# Autodesk Inventor assembly: robot4
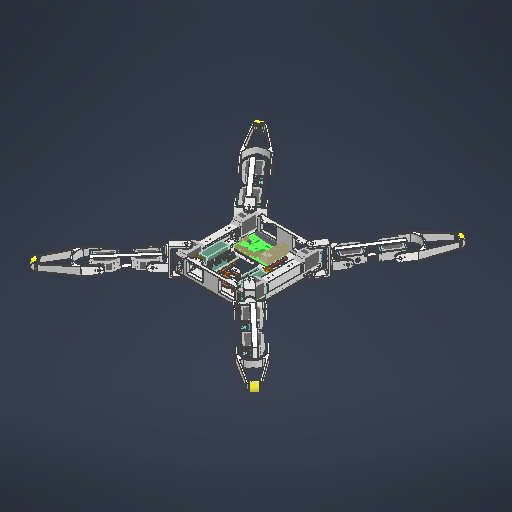
[picture p0: Inventor's stored thumbnail of the model, 512x512]
Saved by Autodesk Inventor 2026.1 (Build 301233000, 233)
## iProperties
Created: 2025-11-03
Part Number: robot4
Document SubType Name: Assembly
Designer: emanuel
Author: emanuel
## Documents named in this file (22)
- C:\Users\emanuel\UnFolder\SpiderRobo\3dmodel\robot6.iam
- C:\Users\emanuel\UnFolder\SpiderRobo\3dmodel\rigid_support1.ipt
- C:\Users\emanuel\UnFolder\SpiderRobo\3dmodel\mg996r.ipt
- C:\Users\emanuel\UnFolder\SpiderRobo\3dmodel\servo_support_4.ipt
- C:\Users\emanuel\UnFolder\SpiderRobo\3dmodel\servo_disc.ipt
- C:\Users\emanuel\UnFolder\SpiderRobo\3dmodel\C1.ipt
- C:\Users\emanuel\UnFolder\SpiderRobo\3dmodel\back_plate.ipt
- C:\Users\emanuel\UnFolder\SpiderRobo\3dmodel\smart_calf.ipt
- C:\Users\emanuel\UnFolder\SpiderRobo\3dmodel\back_servo_support.ipt
- C:\Users\emanuel\UnFolder\SpiderRobo\3dmodel\C2.ipt
- C:\Users\emanuel\UnFolder\SpiderRobo\3dmodel\femur.ipt
- C:\Users\emanuel\UnFolder\SpiderRobo\3dmodel\shoe.ipt
- C:\Users\emanuel\UnFolder\SpiderRobo\3dmodel\shoe_lace.ipt
- C:\Users\emanuel\UnFolder\SpiderRobo\3dmodel\support_2_servo_wide.ipt
- C:\Users\emanuel\UnFolder\SpiderRobo\3dmodel\middle_base.ipt
- C:\Users\emanuel\UnFolder\SpiderRobo\3dmodel\servo_support_4_interior.ipt
- C:\Users\emanuel\UnFolder\SpiderRobo\3dmodel\side_wall1.ipt
- C:\Users\emanuel\UnFolder\SpiderRobo\3dmodel\side_wall2.ipt
- C:\Users\emanuel\UnFolder\SpiderRobo\3dmodel\servo_driver.ipt
- C:\Users\emanuel\UnFolder\SpiderRobo\3dmodel\electronics_holder3.ipt
- C:\Users\emanuel\UnFolder\SpiderRobo\3dmodel\electronics_holder.ipt
- C:\Users\emanuel\UnFolder\SpiderRobo\3dmodel\RaspberryPi5.ipt
## Components (92 placed, 21 different names)
1. rigid_support1:1 — Flush:7, Flush:18, Mate:299, Flush:28, Flush:42, Flush:43, Mate:352, Mate:357
2. rigid_support1:2 — Flush:7, Flush:19, Mate:303, Flush:29, Flush:38, Flush:39, Mate:353
3. mg996r:1 — Mate:7, Mate:8, Mate:20, Mate:21, Mate:251, Mate:301
4. servo_support_4:3 — Flush:1, Flush:3, Flush:24, Flush:25, Mate:301, Mate:342
5. servo_support_4:4 — Flush:1, Mate:7, Mate:8, Flush:26, Flush:27
6. mg996r:2 — Mate:22, Mate:23, Mate:257, Mate:302, Mate:343
7. servo_support_4:5 — Flush:22, Flush:23, Mate:302, Mate:344
8. servo_support_4:6 — Flush:3, Mate:300, Flush:20, Flush:21
9. servo_disc:1 — Mate:20, Mate:21, Mate:250
10. servo_disc:2 — Mate:22, Mate:23, Mate:256
11. mg996r:3 — Mate:247, Mate:298
12. servo_support_4:7 — Mate:298, Flush:32, Flush:36, Mate:339, Flush:47
13. servo_support_4:8 — Mate:304, Flush:30, Flush:31, Mate:321, Flush:44, Flush:45
14. mg996r:4 — Mate:249, Mate:297
15. servo_support_4:10 — Mate:297, Flush:35, Flush:37, Mate:322, Flush:46, Mate:323
16. servo_disc:3 — Mate:246
17. servo_disc:4 — Mate:248
18. back_plate:1
19. smart_calf:1 — Mate:128, Mate:129, Mate:273, Mate:274, Mate:275
20. servo_disc:7 — Mate:128
21. back_servo_support:3
22. C2:2 — Mate:130, Mate:131, Mate:132, Mate:133, Mate:134
23. femur:2
24. mg996r:7 — Mate:129
25. servo_disc:8
26. mg996r:8
27. back_servo_support:4
28. servo_support_4:16
29. servo_support_4:17
30. servo_support_4:18
31. servo_support_4:19
32. C1:1 — Mate:130, Mate:131, Mate:132, Mate:133, Mate:134, Mate:248, Mate:249
33. smart_calf:2 — Mate:289, Mate:290, Mate:291
34. servo_disc:9
35. back_servo_support:5
36. C2:3
37. femur:3
38. mg996r:9
39. servo_disc:10
40. mg996r:10
41. back_servo_support:6
42. servo_support_4:20
43. servo_support_4:21
44. servo_support_4:22
45. servo_support_4:23
46. C1:2 — Mate:256, Mate:257
47. smart_calf:3 — Mate:288, Mate:292, Mate:293
48. servo_disc:11
49. back_servo_support:7
50. C2:4
51. femur:4
52. mg996r:11
53. servo_disc:12
54. mg996r:12
55. back_servo_support:8
56. servo_support_4:24
57. servo_support_4:25
58. servo_support_4:26
59. servo_support_4:27
60. C1:3 — Mate:250, Mate:251
61. smart_calf:4 — Mate:285, Mate:286, Mate:287
62. servo_disc:13
63. back_servo_support:9
64. C2:5
65. femur:5
66. mg996r:13
67. servo_disc:14
68. mg996r:14
69. back_servo_support:10
70. servo_support_4:28
71. servo_support_4:29
72. servo_support_4:30
73. servo_support_4:31
74. C1:4 — Mate:246, Mate:247
75. shoe:1 — Mate:273, Mate:274, Mate:275, Mate:276, Mate:277, Mate:278
76. shoe_lace:1 — Mate:276, Mate:277, Mate:278
77. shoe:2 — Mate:285, Mate:286, Mate:287
78. shoe:3 — Mate:289, Mate:290, Mate:291
79. shoe:4 — Mate:288, Mate:292, Mate:293
80. support_2_servo_wide:2 — Flush:18, Flush:19, Mate:299, Mate:300, Flush:20, Flush:21, Flush:22, Flush:23, Flush:24, Flush:25, Flush:26, Flush:27
81. support_2_servo_wide:3 — Mate:303, Flush:28, Flush:29, Mate:304, Flush:30, Flush:31, Flush:32, Flush:35, Flush:36, Flush:37, Mate:305, Mate:306, Mate:307, Flush:38, Flush:39, Mate:314, Flush:40, Flush:41, Flush:42, Flush:43
82. middle_base:1 — Mate:305, Mate:306, Mate:307, Mate:354, Mate:355, Mate:356
83. servo_support_4_interior:1 — Mate:314, Flush:40, Flush:41, Mate:340, Mate:341
84. side_wall2:1 — Mate:321, Flush:44, Flush:45
85. side_wall2:2 — Mate:322, Flush:46, Mate:323
86. servo_driver:2 — Mate:349, Mate:350, Mate:351
87. servo_driver:3 — Mate:345, Mate:346, Mate:347, Mate:348
88. side_wall1:1 — Mate:339, Flush:47, Mate:340, Mate:341
89. side_wall1:2 — Mate:342, Mate:343, Mate:344
90. electronics_holder:1 — Mate:345, Mate:346, Mate:347, Mate:348, Mate:349, Mate:350, Mate:351, Mate:352, Mate:353, Mate:354
91. RaspberryPi5:1 — Mate:358, Mate:359, Mate:360
92. electronics_holder3:1 — Mate:355, Mate:356, Mate:357, Mate:358, Mate:359, Mate:360
## Relationships (258: Mate 224, Flush 34)
- Flush:1: servo_support_4:3 ↔ servo_support_4:4
- Mate:7: mg996r:1 ↔ servo_support_4:4
- Mate:8: mg996r:1 ↔ servo_support_4:4
- [Flush]: servo_support_4:5 ↔ servo_support_4:6
- [Mate]: mg996r:2 ↔ servo_support_4:6
- [Mate]: mg996r:2 ↔ servo_support_4:6
- Flush:3: servo_support_4:3 ↔ servo_support_4:6
- Mate:20: mg996r:1 ↔ servo_disc:1
- Mate:21: mg996r:1 ↔ servo_disc:1
- Mate:22: mg996r:2 ↔ servo_disc:2
- Mate:23: mg996r:2 ↔ servo_disc:2
- [Flush]: servo_support_4:7 ↔ servo_support_4:8
- [Mate]: mg996r:3 ↔ servo_support_4:8
- [Mate]: mg996r:3 ↔ servo_support_4:8
- [Mate]: mg996r:4 ↔ servo_support_4:10
- [Mate]: mg996r:4 ↔ servo_support_4:10
- [Flush]: servo_support_4:7 ↔ servo_support_4:10
- [Mate]: mg996r:3 ↔ servo_disc:3
- [Mate]: mg996r:3 ↔ servo_disc:3
- [Mate]: mg996r:4 ↔ servo_disc:4
- [Mate]: mg996r:4 ↔ servo_disc:4
- Flush:7: rigid_support1:1 ↔ rigid_support1:2
- [Mate]: servo_disc:7 ↔ mg996r:7
- [Mate]: servo_disc:7 ↔ mg996r:7
- [Mate]: servo_disc:8 ↔ mg996r:8
- [Mate]: servo_disc:8 ↔ mg996r:8
- [Mate]: femur:2 ↔ mg996r:8
- [Mate]: femur:2 ↔ mg996r:8
- [Mate]: femur:2 ↔ mg996r:8
- [Mate]: femur:2 ↔ mg996r:7
- [Mate]: femur:2 ↔ mg996r:7
- [Mate]: femur:2 ↔ mg996r:7
- [Mate]: C2:2 ↔ servo_disc:8
- [Mate]: C2:2 ↔ mg996r:8
- [Mate]: femur:2 ↔ servo_support_4:16
- [Mate]: femur:2 ↔ servo_support_4:19
- [Mate]: femur:2 ↔ servo_support_4:17
- [Mate]: femur:2 ↔ servo_support_4:18
- [Mate]: femur:2 ↔ servo_support_4:16
- [Mate]: mg996r:7 ↔ servo_support_4:19
- [Mate]: back_servo_support:4 ↔ servo_support_4:16
- [Mate]: back_servo_support:4 ↔ servo_support_4:16
- [Mate]: back_servo_support:4 ↔ servo_support_4:16
- [Mate]: back_servo_support:4 ↔ servo_support_4:19
- [Mate]: femur:2 ↔ servo_support_4:16
- [Mate]: femur:2 ↔ servo_support_4:18
- [Mate]: femur:2 ↔ servo_support_4:18
- [Mate]: mg996r:8 ↔ servo_support_4:17
- [Mate]: back_servo_support:3 ↔ servo_support_4:18
- [Mate]: back_servo_support:3 ↔ servo_support_4:18
- [Mate]: back_servo_support:3 ↔ servo_support_4:18
- [Mate]: back_servo_support:3 ↔ servo_support_4:17
- Mate:128: smart_calf:1 ↔ servo_disc:7
- Mate:129: smart_calf:1 ↔ mg996r:7
- Mate:130: C2:2 ↔ C1:1
- Mate:131: C2:2 ↔ C1:1
- Mate:132: C2:2 ↔ C1:1
- Mate:133: C2:2 ↔ C1:1
- Mate:134: C2:2 ↔ C1:1
- [Mate]: servo_disc:9 ↔ mg996r:9
- [Mate]: servo_disc:9 ↔ mg996r:9
- [Mate]: servo_disc:10 ↔ mg996r:10
- [Mate]: servo_disc:10 ↔ mg996r:10
- [Mate]: femur:3 ↔ mg996r:10
- [Mate]: femur:3 ↔ mg996r:10
- [Mate]: femur:3 ↔ mg996r:10
- [Mate]: femur:3 ↔ mg996r:9
- [Mate]: femur:3 ↔ mg996r:9
- [Mate]: femur:3 ↔ mg996r:9
- [Mate]: C2:3 ↔ servo_disc:10
- [Mate]: C2:3 ↔ mg996r:10
- [Mate]: femur:3 ↔ servo_support_4:20
- [Mate]: femur:3 ↔ servo_support_4:23
- [Mate]: femur:3 ↔ servo_support_4:21
- [Mate]: femur:3 ↔ servo_support_4:22
- [Mate]: femur:3 ↔ servo_support_4:20
- [Mate]: mg996r:9 ↔ servo_support_4:23
- [Mate]: back_servo_support:6 ↔ servo_support_4:20
- [Mate]: back_servo_support:6 ↔ servo_support_4:20
- [Mate]: back_servo_support:6 ↔ servo_support_4:20
- [Mate]: back_servo_support:6 ↔ servo_support_4:23
- [Mate]: femur:3 ↔ servo_support_4:20
- [Mate]: femur:3 ↔ servo_support_4:22
- [Mate]: femur:3 ↔ servo_support_4:22
- [Mate]: mg996r:10 ↔ servo_support_4:21
- [Mate]: back_servo_support:5 ↔ servo_support_4:22
- [Mate]: back_servo_support:5 ↔ servo_support_4:22
- [Mate]: back_servo_support:5 ↔ servo_support_4:22
- [Mate]: back_servo_support:5 ↔ servo_support_4:21
- [Mate]: smart_calf:2 ↔ servo_disc:9
- [Mate]: smart_calf:2 ↔ mg996r:9
- [Mate]: C2:3 ↔ C1:2
- [Mate]: C2:3 ↔ C1:2
- [Mate]: C2:3 ↔ C1:2
- [Mate]: C2:3 ↔ C1:2
- [Mate]: C2:3 ↔ C1:2
- [Mate]: servo_disc:11 ↔ mg996r:11
- [Mate]: servo_disc:11 ↔ mg996r:11
- [Mate]: servo_disc:12 ↔ mg996r:12
- [Mate]: servo_disc:12 ↔ mg996r:12
- [Mate]: femur:4 ↔ mg996r:12
- [Mate]: femur:4 ↔ mg996r:12
- [Mate]: femur:4 ↔ mg996r:12
- [Mate]: femur:4 ↔ mg996r:11
- [Mate]: femur:4 ↔ mg996r:11
- [Mate]: femur:4 ↔ mg996r:11
- [Mate]: C2:4 ↔ servo_disc:12
- [Mate]: C2:4 ↔ mg996r:12
- [Mate]: femur:4 ↔ servo_support_4:24
- [Mate]: femur:4 ↔ servo_support_4:27
- [Mate]: femur:4 ↔ servo_support_4:25
- [Mate]: femur:4 ↔ servo_support_4:26
- [Mate]: femur:4 ↔ servo_support_4:24
- [Mate]: mg996r:11 ↔ servo_support_4:27
- [Mate]: back_servo_support:8 ↔ servo_support_4:24
- [Mate]: back_servo_support:8 ↔ servo_support_4:24
- [Mate]: back_servo_support:8 ↔ servo_support_4:24
- [Mate]: back_servo_support:8 ↔ servo_support_4:27
- [Mate]: femur:4 ↔ servo_support_4:24
- [Mate]: femur:4 ↔ servo_support_4:26
- [Mate]: femur:4 ↔ servo_support_4:26
- [Mate]: mg996r:12 ↔ servo_support_4:25
- [Mate]: back_servo_support:7 ↔ servo_support_4:26
- [Mate]: back_servo_support:7 ↔ servo_support_4:26
- [Mate]: back_servo_support:7 ↔ servo_support_4:26
- [Mate]: back_servo_support:7 ↔ servo_support_4:25
- [Mate]: smart_calf:3 ↔ servo_disc:11
- [Mate]: smart_calf:3 ↔ mg996r:11
- [Mate]: C2:4 ↔ C1:3
- [Mate]: C2:4 ↔ C1:3
- [Mate]: C2:4 ↔ C1:3
- [Mate]: C2:4 ↔ C1:3
- [Mate]: C2:4 ↔ C1:3
- [Mate]: servo_disc:13 ↔ mg996r:13
- [Mate]: servo_disc:13 ↔ mg996r:13
- [Mate]: servo_disc:14 ↔ mg996r:14
- [Mate]: servo_disc:14 ↔ mg996r:14
- [Mate]: femur:5 ↔ mg996r:14
- [Mate]: femur:5 ↔ mg996r:14
- [Mate]: femur:5 ↔ mg996r:14
- [Mate]: femur:5 ↔ mg996r:13
- [Mate]: femur:5 ↔ mg996r:13
- [Mate]: femur:5 ↔ mg996r:13
- [Mate]: C2:5 ↔ servo_disc:14
- [Mate]: C2:5 ↔ mg996r:14
- [Mate]: femur:5 ↔ servo_support_4:28
- [Mate]: femur:5 ↔ servo_support_4:31
- [Mate]: femur:5 ↔ servo_support_4:29
- [Mate]: femur:5 ↔ servo_support_4:30
- [Mate]: femur:5 ↔ servo_support_4:28
- [Mate]: mg996r:13 ↔ servo_support_4:31
- [Mate]: back_servo_support:10 ↔ servo_support_4:28
- [Mate]: back_servo_support:10 ↔ servo_support_4:28
- [Mate]: back_servo_support:10 ↔ servo_support_4:28
- [Mate]: back_servo_support:10 ↔ servo_support_4:31
- [Mate]: femur:5 ↔ servo_support_4:28
- [Mate]: femur:5 ↔ servo_support_4:30
- [Mate]: femur:5 ↔ servo_support_4:30
- [Mate]: mg996r:14 ↔ servo_support_4:29
- [Mate]: back_servo_support:9 ↔ servo_support_4:30
- [Mate]: back_servo_support:9 ↔ servo_support_4:30
- [Mate]: back_servo_support:9 ↔ servo_support_4:30
- [Mate]: back_servo_support:9 ↔ servo_support_4:29
- [Mate]: smart_calf:4 ↔ servo_disc:13
- [Mate]: smart_calf:4 ↔ mg996r:13
- [Mate]: C2:5 ↔ C1:4
- [Mate]: C2:5 ↔ C1:4
- [Mate]: C2:5 ↔ C1:4
- [Mate]: C2:5 ↔ C1:4
- [Mate]: C2:5 ↔ C1:4
- Mate:246: servo_disc:3 ↔ C1:4
- Mate:247: mg996r:3 ↔ C1:4
- Mate:248: servo_disc:4 ↔ C1:1
- Mate:249: mg996r:4 ↔ C1:1
- Mate:250: servo_disc:1 ↔ C1:3
- Mate:251: mg996r:1 ↔ C1:3
- Mate:256: servo_disc:2 ↔ C1:2
- Mate:257: mg996r:2 ↔ C1:2
- Mate:273: smart_calf:1 ↔ shoe:1
- Mate:274: smart_calf:1 ↔ shoe:1
- Mate:275: smart_calf:1 ↔ shoe:1
- Mate:276: shoe:1 ↔ shoe_lace:1
- Mate:277: shoe:1 ↔ shoe_lace:1
- Mate:278: shoe:1 ↔ shoe_lace:1
- Mate:285: smart_calf:4 ↔ shoe:2
- Mate:286: smart_calf:4 ↔ shoe:2
- Mate:287: smart_calf:4 ↔ shoe:2
- Mate:288: smart_calf:3 ↔ shoe:4
- Mate:289: smart_calf:2 ↔ shoe:3
- Mate:290: smart_calf:2 ↔ shoe:3
- Mate:291: smart_calf:2 ↔ shoe:3
- Mate:292: smart_calf:3 ↔ shoe:4
- Mate:293: smart_calf:3 ↔ shoe:4
- Mate:297 (4 mm): mg996r:4 ↔ servo_support_4:10
- Mate:298 (4 mm): mg996r:3 ↔ servo_support_4:7
- Flush:18: rigid_support1:1 ↔ support_2_servo_wide:2
- Flush:19: rigid_support1:2 ↔ support_2_servo_wide:2
- Mate:299: rigid_support1:1 ↔ support_2_servo_wide:2
- Mate:300: servo_support_4:6 ↔ support_2_servo_wide:2
- Flush:20: servo_support_4:6 ↔ support_2_servo_wide:2
- Flush:21: servo_support_4:6 ↔ support_2_servo_wide:2
- Flush:22: servo_support_4:5 ↔ support_2_servo_wide:2
- Flush:23: servo_support_4:5 ↔ support_2_servo_wide:2
- Flush:24: servo_support_4:3 ↔ support_2_servo_wide:2
- Flush:25: servo_support_4:3 ↔ support_2_servo_wide:2
- Flush:26: servo_support_4:4 ↔ support_2_servo_wide:2
- Flush:27: servo_support_4:4 ↔ support_2_servo_wide:2
- Mate:301 (4 mm): mg996r:1 ↔ servo_support_4:3
- Mate:302 (4 mm): mg996r:2 ↔ servo_support_4:5
- Mate:303: rigid_support1:2 ↔ support_2_servo_wide:3
- Flush:28: rigid_support1:1 ↔ support_2_servo_wide:3
- Flush:29: rigid_support1:2 ↔ support_2_servo_wide:3
- Mate:304: servo_support_4:8 ↔ support_2_servo_wide:3
- Flush:30: servo_support_4:8 ↔ support_2_servo_wide:3
- Flush:31: servo_support_4:8 ↔ support_2_servo_wide:3
- Flush:32: servo_support_4:7 ↔ support_2_servo_wide:3
- Flush:35: servo_support_4:10 ↔ support_2_servo_wide:3
- Flush:36: servo_support_4:7 ↔ support_2_servo_wide:3
- Flush:37: servo_support_4:10 ↔ support_2_servo_wide:3
- Mate:305: support_2_servo_wide:3 ↔ middle_base:1
- Mate:306: support_2_servo_wide:3 ↔ middle_base:1
- Mate:307: support_2_servo_wide:3 ↔ middle_base:1
- Flush:38: rigid_support1:2 ↔ support_2_servo_wide:3
- Flush:39: rigid_support1:2 ↔ support_2_servo_wide:3
- Mate:314: support_2_servo_wide:3 ↔ servo_support_4_interior:1
- Flush:40: support_2_servo_wide:3 ↔ servo_support_4_interior:1
- Flush:41: support_2_servo_wide:3 ↔ servo_support_4_interior:1
- Flush:42: rigid_support1:1 ↔ support_2_servo_wide:3
- Flush:43: rigid_support1:1 ↔ support_2_servo_wide:3
- Mate:321: servo_support_4:8 ↔ side_wall2:1
- Flush:44: servo_support_4:8 ↔ side_wall2:1
- Flush:45: servo_support_4:8 ↔ side_wall2:1
- Mate:322: servo_support_4:10 ↔ side_wall2:2
- Flush:46: servo_support_4:10 ↔ side_wall2:2
- Mate:323: servo_support_4:10 ↔ side_wall2:2
- Mate:339: servo_support_4:7 ↔ side_wall1:1
- Flush:47: servo_support_4:7 ↔ side_wall1:1
- Mate:340: servo_support_4_interior:1 ↔ side_wall1:1
- Mate:341: servo_support_4_interior:1 ↔ side_wall1:1
- Mate:342: servo_support_4:3 ↔ side_wall1:2
- Mate:343: mg996r:2 ↔ side_wall1:2
- Mate:344: servo_support_4:5 ↔ side_wall1:2
- Mate:345: servo_driver:3 ↔ electronics_holder:1
- Mate:346: servo_driver:3 ↔ electronics_holder:1
- Mate:347: servo_driver:3 ↔ electronics_holder:1
- Mate:348: servo_driver:3 ↔ electronics_holder:1
- Mate:349: servo_driver:2 ↔ electronics_holder:1
- Mate:350: servo_driver:2 ↔ electronics_holder:1
- Mate:351: servo_driver:2 ↔ electronics_holder:1
- Mate:352: rigid_support1:1 ↔ electronics_holder:1
- Mate:353: rigid_support1:2 ↔ electronics_holder:1
- Mate:354: middle_base:1 ↔ electronics_holder:1
- Mate:355: middle_base:1 ↔ electronics_holder3:1
- Mate:356: middle_base:1 ↔ electronics_holder3:1
- Mate:357: rigid_support1:1 ↔ electronics_holder3:1
- Mate:358: RaspberryPi5:1 ↔ electronics_holder3:1
- Mate:359: RaspberryPi5:1 ↔ electronics_holder3:1
- Mate:360: RaspberryPi5:1 ↔ electronics_holder3:1
## Named parameters: d24_d19 = 0 mm, d25_d22 = 0 mm, d26_d23 = 0 mm, d45_d19 = 0 mm, d48_d22 = 0 mm, d49_d23 = 0 mm, d51_d25_d22 = 0 mm, d52_d26_d23 = 0 mm, d59_d33 = 0 mm, d63_d37 = 0 mm, d64_d38 = 0 mm, d65_d39 = 0 mm, d66_d40 = 0 mm, d125_d101 = 0 mm, d126_d102 = 0 mm, d127_d103 = 0 mm, d128_d104 = 0 mm, d129_d105 = 0 mm, d130_d106 = 0 mm, d131_d107 = 0 mm, d132_d108 = 0 mm, d133_d109 = 0 mm, d134_d110 = 0 mm, d135_d111 = 0 mm, d136_d112 = 0 mm, d137_d113 = 0 mm, d138_d114 = 0 mm, d139_d115 = 0 mm, d140_d116 = 0 mm, d141_d117 = 0 mm, d142_d118 = 0 mm, d143_d119 = 0 mm, d144_d120 = 0 mm, d145_d121 = 0 mm, d146_d122 = 0 mm, d147_d123 = 0 mm, d148_d124 = 0 mm, d149_d95 = 0 mm, d150_d96 = 0 mm, d151_d97_d95 = 0 mm, d152_d98_d96 = 0 mm, d153_d99 = 0 mm, d154_d100 = 0 mm, d231_d226 = 0 mm, d232_d227 = 0 mm, d233_d228 = 0 mm, d234_d229 = 0 mm, d235_d155 = 0 mm, d236_d156 = 0 mm, d237_d125_d101 = 0 mm, d238_d126_d102 = 0 mm, d239_d127_d103 = 0 mm, d240_d128_d104 = 0 mm, d241_d129_d105 = 0 mm, d242_d130_d106 = 0 mm, d243_d131_d107 = 0 mm, d244_d132_d108 = 0 mm, d245_d133_d109 = 0 mm, d246_d134_d110 = 0 mm, d247_d135_d111 = 0 mm, d248_d136_d112 = 0 mm, d249_d137_d113 = 0 mm, d250_d138_d114 = 0 mm, d251_d139_d115 = 0 mm, d252_d140_d116 = 0 mm, d253_d141_d117 = 0 mm, d254_d142_d118 = 0 mm, d255_d143_d119 = 0 mm, d256_d144_d120 = 0 mm, d257_d145_d121 = 0 mm, d258_d146_d122 = 0 mm, d259_d147_d123 = 0 mm, d260_d148_d124 = 0 mm, d261_d149_d95 = 0 mm, d262_d150_d96 = 0 mm, d263_d151_d97_d95 = 0 mm, d264_d152_d98_d96 = 0 mm, d265_d153_d99 = 0 mm, d266_d154_d100 = 0 mm, d267_d230 = 0 mm, d268_d226 = 0 mm, d269_d227 = 0 mm, d270_d228 = 0 mm, d271_d229 = 0 mm, d272_d155 = 0 mm, d273_d156 = 0 mm, d274_d125_d101 = 0 mm, d275_d126_d102 = 0 mm, d276_d127_d103 = 0 mm, d277_d128_d104 = 0 mm, d278_d129_d105 = 0 mm, d279_d130_d106 = 0 mm, d280_d131_d107 = 0 mm, d281_d132_d108 = 0 mm, d282_d133_d109 = 0 mm, d283_d134_d110 = 0 mm, d284_d135_d111 = 0 mm, d285_d136_d112 = 0 mm, d286_d137_d113 = 0 mm, d287_d138_d114 = 0 mm, d288_d139_d115 = 0 mm, d289_d140_d116 = 0 mm, d290_d141_d117 = 0 mm, d291_d142_d118 = 0 mm, d292_d143_d119 = 0 mm, d293_d144_d120 = 0 mm, d294_d145_d121 = 0 mm, d295_d146_d122 = 0 mm, d296_d147_d123 = 0 mm, d297_d148_d124 = 0 mm, d298_d149_d95 = 0 mm, d299_d150_d96 = 0 mm, d300_d151_d97_d95 = 0 mm, d301_d152_d98_d96 = 0 mm, d302_d153_d99 = 0 mm, d303_d154_d100 = 0 mm, d304_d230 = 0 mm, d305_d226 = 0 mm, d306_d227 = 0 mm, d307_d228 = 0 mm, d308_d229 = 0 mm, d309_d155 = 0 mm, d310_d156 = 0 mm, d311_d125_d101 = 0 mm, d312_d126_d102 = 0 mm, d313_d127_d103 = 0 mm, d314_d128_d104 = 0 mm, d315_d129_d105 = 0 mm, d316_d130_d106 = 0 mm, d317_d131_d107 = 0 mm, d318_d132_d108 = 0 mm, d319_d133_d109 = 0 mm, d320_d134_d110 = 0 mm, d321_d135_d111 = 0 mm, d322_d136_d112 = 0 mm, d323_d137_d113 = 0 mm, d324_d138_d114 = 0 mm, d325_d139_d115 = 0 mm, d326_d140_d116 = 0 mm, d327_d141_d117 = 0 mm, d328_d142_d118 = 0 mm, d329_d143_d119 = 0 mm, d330_d144_d120 = 0 mm, d331_d145_d121 = 0 mm, d332_d146_d122 = 0 mm, d333_d147_d123 = 0 mm, d334_d148_d124 = 0 mm, d335_d149_d95 = 0 mm, d336_d150_d96 = 0 mm, d337_d151_d97_d95 = 0 mm, d338_d152_d98_d96 = 0 mm, d339_d153_d99 = 0 mm, d340_d154_d100 = 0 mm, d341_d230 = 0 mm
